# Autodesk Inventor assembly: GearboxAssembly
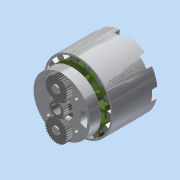
[picture p0: Inventor's stored thumbnail of the model, 180x180]
Saved by Autodesk Inventor 2015 (Build 190159000, 159)
## iProperties
Created: 2015-12-24
Part Number: GearboxAssembly
Document SubType Name: Assembly
Designer: Raphael
Author: Raphael
## Documents named in this file (6)
- \\psf\Home\Documents\electric-skateboard\CAD\HubMotor\GearboxAssembly.iam
- \\psf\Home\Documents\electric-skateboard\CAD\HubMotor\StatorAssembly.iam
- \\psf\Home\Documents\electric-skateboard\CAD\HubMotor\RotorAssembly.iam
- \\psf\Home\Documents\electric-skateboard\CAD\HubMotor\PlanetaryAssembly.iam
- \\psf\Home\Documents\electric-skateboard\CAD\HubMotor\SunGear.ipt
- \\psf\Home\Documents\electric-skateboard\CAD\HubMotor\M15Bearing.ipt
## Components (6 placed, 5 different names)
1. StatorAssembly:1 [sub-assembly] — Mate:1, Mate:2, Flush:1, Mate:3, Mate:8, Mate:9, Mate:10
2. RotorAssembly:1 [sub-assembly] — Mate:1, Mate:4, Mate:5, Mate:6, Mate:7
3. PlanetaryAssembly:1 [sub-assembly] — Mate:7, Mate:8, Mate:9
4. SunGear:1 — Mate:5, Mate:6
5. M15Bearing:2 — Mate:2, Flush:1, Mate:4
6. M15Bearing:3 — Mate:3, Mate:10
## Relationships (11: Mate 10, Flush 1)
- Mate:1: StatorAssembly:1 ↔ RotorAssembly:1
- Mate:2: StatorAssembly:1 ↔ M15Bearing:2
- Flush:1: StatorAssembly:1 ↔ M15Bearing:2
- Mate:3: StatorAssembly:1 ↔ M15Bearing:3
- Mate:4: RotorAssembly:1 ↔ M15Bearing:2
- Mate:5: RotorAssembly:1 ↔ SunGear:1
- Mate:6: RotorAssembly:1 ↔ SunGear:1
- Mate:7: RotorAssembly:1 ↔ PlanetaryAssembly:1
- Mate:8: StatorAssembly:1 ↔ PlanetaryAssembly:1
- Mate:9: StatorAssembly:1 ↔ PlanetaryAssembly:1
- Mate:10: StatorAssembly:1 ↔ M15Bearing:3
